# Autodesk Inventor assembly: ASM_Micron_ASAP_Merge2
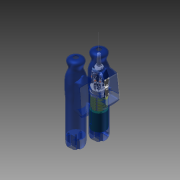
[picture p0: Inventor's stored thumbnail of the model, 180x180]
Saved by Autodesk Inventor 2011 SP2 (Build 150309200, 309)
## iProperties
Created: 2011-10-07
Part Number: ASM_Micron_ASAP_Merge2
Document SubType Name: Assembly
Designer: sungwook
Author: sungwook
## Documents named in this file (26)
- C:\Users\sungwook\Documents\Inventor\Micron20\Assembly\Motion_Merge\ASM_Micron_ASAP_Merge2.iam
- C:\Users\sungwook\Documents\Inventor\Micron20\Assembly\Motion_Merge\ASM_Micron_ASAP_Indep0.iam
- C:\Users\sungwook\Documents\Inventor\Micron20\Assembly\Motion_Merge\ASM_Micron_ASAP_Indep10.iam
- C:\Users\sungwook\Documents\Inventor\Micron20\Assembly\Motion_Merge\ASM_Micron_ASAP_Indep20.iam
- C:\Users\sungwook\Documents\Inventor\Micron20\Assembly\Motion_Merge\ASM_Micron_ASAP_Indep30.iam
- C:\Users\sungwook\Documents\Inventor\Micron20\Assembly\Motion_Merge\ASM_Micron_ASAP_Indep40.iam
- C:\Users\sungwook\Documents\Inventor\Micron20\Assembly\Motion_Merge\ASM_Micron_ASAP_Indep50.iam
- C:\Users\sungwook\Documents\Inventor\Micron20\Assembly\Motion_Merge\ASM_Micron_ASAP_Indep60.iam
- C:\Users\sungwook\Documents\Inventor\Micron20\Assembly\Motion_Merge\ASM_Micron_ASAP_Indep70.iam
- C:\Users\sungwook\Documents\Inventor\Micron20\Assembly\Motion_Merge\ASM_Micron_ASAP_Indep80.iam
- C:\Users\sungwook\Documents\Inventor\Micron20\Assembly\Motion_Merge\ASM_Micron_ASAP_Indep90.iam
- C:\Users\sungwook\Documents\Inventor\Micron20\Assembly\Motion_Merge\ASM_Micron_ASAP_Indep100.iam
- C:\Users\sungwook\Documents\Inventor\Micron20\Assembly\Motion_Merge\ASM_Micron_ASAP_Indep110.iam
- C:\Users\sungwook\Documents\Inventor\Micron20\Assembly\Motion_Merge\ASM_Micron_ASAP_Indep120.iam
- C:\Users\sungwook\Documents\Inventor\Micron20\Assembly\Motion_Merge\ASM_Micron_ASAP_Indep130.iam
- C:\Users\sungwook\Documents\Inventor\Micron20\Assembly\Motion_Merge\ASM_Micron_ASAP_Indep140.iam
- C:\Users\sungwook\Documents\Inventor\Micron20\Parts\Handle\ex\Case6.ipt
- C:\Users\sungwook\Documents\Inventor\Micron20\Parts\ASAP\Handle_ASAP.iam
- C:\Users\sungwook\Documents\Inventor\Micron20\Parts\Electronics\PCB_Stack.iam
- C:\Users\sungwook\Documents\Inventor\Micron20\Parts\Handle\Handle_1_rev.ipt
- C:\Users\sungwook\Documents\Inventor\Micron20\Parts\Handle\Handle_1_rev_Head.ipt
- C:\Users\sungwook\Documents\Inventor\Micron20\Parts\Handle\Handle_1_rev_Back.ipt
- C:\Users\sungwook\Documents\Inventor\Micron20\Parts\Handle\Handle_1_rev_Back_part1.ipt
- C:\Users\sungwook\Documents\Inventor\Micron20\Parts\Handle\Handle_1_rev_Back_part2.ipt
- C:\Users\sungwook\Documents\Inventor\Micron20\Parts\Handle\Window.ipt
- C:\Users\sungwook\Documents\Inventor\Micron20\Parts\Handle\Handle_2.ipt
## Components (25 placed, 25 different names)
1. (0,0,0) [sub-assembly] — Flush:2, Mate:2, Flush:4, Flush:6, Flush:8, Flush:10, Flush:12, Flush:14, Flush:16, Flush:18, Flush:21, Flush:24, Flush:26, Flush:28, Mate:28, Mate:29, Mate:30, Mate:31, Mate:32, Mate:33, Mate:34, Mate:35, Mate:36, Mate:37, Mate:38, Mate:39, Mate:40, Mate:41, Mate:42, Mate:43, Mate:44, Mate:45, Mate:46, Mate:47, Mate:48, Mate:49, Mate:50, Flush:31, Mate:51, Mate:52, Mate:53, Mate:54, Mate:55, Mate:73, Mate:74, Mate:81, Mate:82, Mate:83, Mate:94
2. (0,2,0) [sub-assembly] — Flush:2, Mate:28, Mate:29
3. pi/2,2,0 [sub-assembly] — Flush:4, Flush:30, Mate:30
4. pi,2,0 [sub-assembly] — Flush:6, Mate:31, Mate:32
5. -pi/2,2,0 [sub-assembly] — Flush:8, Mate:33, Mate:34
6. 0,0,-2 [sub-assembly] — Flush:10, Mate:37, Mate:38
7. 0,2,-2 [sub-assembly] — Flush:12, Mate:39, Mate:40
8. pi/2,2,-2 [sub-assembly] — Flush:21, Mate:41, Mate:42
9. pi,2,-2 [sub-assembly] — Flush:16, Mate:35, Mate:36
10. -pi/2,2,-2 [sub-assembly] — Flush:14, Mate:43, Mate:44
11. 0,0,2 [sub-assembly] — Flush:18, Mate:45, Mate:46
12. 0,2,2 [sub-assembly] — Flush:28, Mate:47, Mate:48
13. pi/2,2,2 [sub-assembly] — Mate:49, Mate:50, Flush:31
14. pi,2,2 [sub-assembly] — Flush:24, Mate:51, Mate:52
15. -pi/2,2,2 [sub-assembly] — Flush:26, Mate:53, Mate:54, Mate:56, Mate:72
16. Case6:1 — Mate:57, Flush:32
17. Handle_ASAP:1 [sub-assembly] — Mate:55, Mate:56
18. PCB_Stack:1 [sub-assembly] — Mate:72, Flush:73, Mate:73, Mate:74
19. Handle_1_rev:1 — Mate:77, Mate:78
20. Handle_1_rev_Head:1 — Mate:80, Mate:81, Mate:82, Mate:83, Mate:86, Mate:87, Flush:88, Mate:88, Mate:89, Mate:90, Mate:91, Mate:92, Mate:95, Mate:97, Mate:98, Mate:99, Mate:100
21. Handle_1_rev_Back:1 — Mate:86, Mate:87, Flush:88, Mate:88, Mate:89
22. Handle_1_rev_Back_part1:1 — Mate:90, Mate:91, Mate:92, Mate:93, Mate:95, Mate:96
23. Handle_1_rev_Back_part2:1 — Mate:93, Mate:94, Mate:96, Mate:97
24. Window:1 — Mate:98, Mate:99, Mate:100
25. Handle_2:1 — Mate:101
## Relationships (74: Mate 56, Flush 18)
- Flush:2: (0,0,0) ↔ (0,2,0)
- Mate:2: (0,0,0)
- Flush:4: (0,0,0) ↔ pi/2,2,0
- Flush:6: (0,0,0) ↔ pi,2,0
- Flush:8: (0,0,0) ↔ -pi/2,2,0
- Flush:10: (0,0,0) ↔ 0,0,-2
- Flush:12: (0,0,0) ↔ 0,2,-2
- Flush:14: (0,0,0) ↔ -pi/2,2,-2
- Flush:16: (0,0,0) ↔ pi,2,-2
- Flush:18: (0,0,0) ↔ 0,0,2
- Flush:21: (0,0,0) ↔ pi/2,2,-2
- Flush:24: (0,0,0) ↔ pi,2,2
- Flush:26: (0,0,0) ↔ -pi/2,2,2
- Flush:28: (0,0,0) ↔ 0,2,2
- Mate:28: (0,0,0) ↔ (0,2,0)
- Mate:29: (0,0,0) ↔ (0,2,0)
- Flush:30: pi/2,2,0
- Mate:30: (0,0,0) ↔ pi/2,2,0
- Mate:31: (0,0,0) ↔ pi,2,0
- Mate:32: (0,0,0) ↔ pi,2,0
- Mate:33: (0,0,0) ↔ -pi/2,2,0
- Mate:34: (0,0,0) ↔ -pi/2,2,0
- Mate:35: (0,0,0) ↔ pi,2,-2
- Mate:36: (0,0,0) ↔ pi,2,-2
- Mate:37: (0,0,0) ↔ 0,0,-2
- Mate:38: (0,0,0) ↔ 0,0,-2
- Mate:39: (0,0,0) ↔ 0,2,-2
- Mate:40: (0,0,0) ↔ 0,2,-2
- Mate:41: (0,0,0) ↔ pi/2,2,-2
- Mate:42: (0,0,0) ↔ pi/2,2,-2
- Mate:43: (0,0,0) ↔ -pi/2,2,-2
- Mate:44: (0,0,0) ↔ -pi/2,2,-2
- Mate:45: (0,0,0) ↔ 0,0,2
- Mate:46: (0,0,0) ↔ 0,0,2
- Mate:47: (0,0,0) ↔ 0,2,2
- Mate:48: (0,0,0) ↔ 0,2,2
- Mate:49: (0,0,0) ↔ pi/2,2,2
- Mate:50: (0,0,0) ↔ pi/2,2,2
- Flush:31: (0,0,0) ↔ pi/2,2,2
- Mate:51: (0,0,0) ↔ pi,2,2
- Mate:52: (0,0,0) ↔ pi,2,2
- Mate:53: (0,0,0) ↔ -pi/2,2,2
- Mate:54: (0,0,0) ↔ -pi/2,2,2
- Mate:55: (0,0,0) ↔ Handle_ASAP:1
- Mate:56: -pi/2,2,2 ↔ Handle_ASAP:1
- Mate:57: Case6:1
- Flush:32: Case6:1
- Mate:72: -pi/2,2,2 ↔ PCB_Stack:1
- Flush:73: PCB_Stack:1
- Mate:73: (0,0,0) ↔ PCB_Stack:1
- Mate:74: (0,0,0) ↔ PCB_Stack:1
- Mate:77: Handle_1_rev:1
- Mate:78: Handle_1_rev:1
- Mate:80: Handle_1_rev_Head:1
- Mate:81: (0,0,0) ↔ Handle_1_rev_Head:1
- Mate:82: (0,0,0) ↔ Handle_1_rev_Head:1
- Mate:83: (0,0,0) ↔ Handle_1_rev_Head:1
- Mate:86: Handle_1_rev_Head:1 ↔ Handle_1_rev_Back:1
- Mate:87: Handle_1_rev_Head:1 ↔ Handle_1_rev_Back:1
- Flush:88: Handle_1_rev_Head:1 ↔ Handle_1_rev_Back:1
- Mate:88: Handle_1_rev_Head:1 ↔ Handle_1_rev_Back:1
- Mate:89: Handle_1_rev_Head:1 ↔ Handle_1_rev_Back:1
- Mate:90: Handle_1_rev_Head:1 ↔ Handle_1_rev_Back_part1:1
- Mate:91: Handle_1_rev_Head:1 ↔ Handle_1_rev_Back_part1:1
- Mate:92: Handle_1_rev_Head:1 ↔ Handle_1_rev_Back_part1:1
- Mate:93: Handle_1_rev_Back_part1:1 ↔ Handle_1_rev_Back_part2:1
- Mate:94: (0,0,0) ↔ Handle_1_rev_Back_part2:1
- Mate:95: Handle_1_rev_Head:1 ↔ Handle_1_rev_Back_part1:1
- Mate:96: Handle_1_rev_Back_part1:1 ↔ Handle_1_rev_Back_part2:1
- Mate:97: Handle_1_rev_Head:1 ↔ Handle_1_rev_Back_part2:1
- Mate:98: Handle_1_rev_Head:1 ↔ Window:1
- Mate:99: Handle_1_rev_Head:1 ↔ Window:1
- Mate:100: Handle_1_rev_Head:1 ↔ Window:1
- Mate:101: Handle_2:1
